# Autodesk Inventor assembly: Assembly1
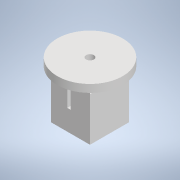
[picture p0: Inventor's stored thumbnail of the model, 180x180]
Saved by Autodesk Inventor 2022 (Build 260153000, 153)
## iProperties
Created: 2022-04-06
Part Number: Assembly1
Document SubType Name: Assembly
Designer: awp
Author: awp
## Documents named in this file (5)
- C:\Rice\Junior\Elec327\FinalProject\Assembly1.iam
- C:\Rice\Junior\Elec327\FinalProject\SpringPotBottom.ipt
- C:\Rice\Junior\Elec327\FinalProject\Knob.ipt
- C:\Rice\Junior\Elec327\FinalProject\Pot.ipt
- C:\Rice\Junior\Elec327\FinalProject\TurnBot.ipt
## Components (4 placed, 4 different names)
1. SpringPotBottom:1 — Mate:1, Flush:1, Mate:2, Mate:3
2. Knob:1 — Mate:1, Mate:6
3. Pot:1 — Flush:1, Mate:2, Mate:3, Mate:4, Mate:5
4. TurnBot:1 — Mate:4, Mate:5, Mate:6
## Relationships (7: Mate 6, Flush 1)
- Mate:1: SpringPotBottom:1 ↔ Knob:1
- Flush:1: SpringPotBottom:1 ↔ Pot:1
- Mate:2: SpringPotBottom:1 ↔ Pot:1
- Mate:3: SpringPotBottom:1 ↔ Pot:1
- Mate:4: Pot:1 ↔ TurnBot:1
- Mate:5: Pot:1 ↔ TurnBot:1
- Mate:6: Knob:1 ↔ TurnBot:1
